# Autodesk Inventor assembly: Shooter Assembly
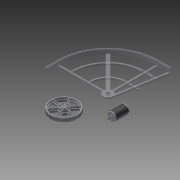
[picture p0: Inventor's stored thumbnail of the model, 180x180]
Saved by Autodesk Inventor 2013 (Build 170138000, 138)
## iProperties
Created: 2013-01-15
Part Number: Shooter Assembly
Document SubType Name: Assembly
Designer: actoennies
Mass: 2159.78 g
Surface Area: 5034.93 cm^2
Volume: 1407.21 cm^3
Density: 1.5348 g/cm^3
Author: actoennies
## Documents named in this file (7)
- H:\Robotics\Shooter\Shooter Assembly.iam
- \\NNHSSRV2.hs.sd203.org\ACToennies$\Robotics\Shooter\Bearing Mount v1.ipt
- \\NNHSSRV2.hs.sd203.org\ACToennies$\Robotics\Shooter\Outer Rail v1.ipt
- \\NNHSSRV2.hs.sd203.org\ACToennies$\Robotics\Shooter\Runner Rails v2.ipt
- \\NNHSSRV2.hs.sd203.org\ACToennies$\Robotics\Parts\1.125 OD .375 ID BEARING\Bearing_AndyMark_am_0209.ipt
- \\NNHSSRV2.hs.sd203.org\ACToennies$\Robotics\Parts\CIM Motor\Motors_FR801-001.iam
- \\NNHSSRV2.hs.sd203.org\ACToennies$\Inventor\8 Plaction Wheel.iam
## Components (6 placed, 6 different names)
1. Bearing Mount v1:1 — Insert:3, Insert:4, Insert:5, Insert:6, Flush:1, Insert:7
2. Outer Rail v1:1 — Insert:3, Insert:4
3. Runner Rails v2:1 — Insert:5, Insert:6
4. Bearing_AndyMark_am_0209:1 — Flush:1, Insert:7
5. Motors_FR801-001:1 [sub-assembly]
6. 8 Plaction Wheel:1 [sub-assembly]
## Relationships (6: Insert 5, Flush 1)
- Insert:3: Bearing Mount v1:1 ↔ Outer Rail v1:1
- Insert:4: Bearing Mount v1:1 ↔ Outer Rail v1:1
- Insert:5: Bearing Mount v1:1 ↔ Runner Rails v2:1
- Insert:6: Bearing Mount v1:1 ↔ Runner Rails v2:1
- Flush:1: Bearing Mount v1:1 ↔ Bearing_AndyMark_am_0209:1
- Insert:7: Bearing Mount v1:1 ↔ Bearing_AndyMark_am_0209:1
